# Autodesk Inventor assembly: Assembly1
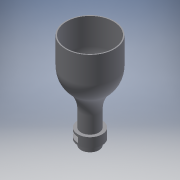
[picture p0: Inventor's stored thumbnail of the model, 180x180]
Saved by Autodesk Inventor 2018.3 (Build 223284000, 284)
## iProperties
Created: 2020-03-27
Part Number: Assembly1
Document SubType Name: Assembly
Designer: ToreDenStore
Author: ToreDenStore
## Documents named in this file (3)
- C:\Users\ToreDenStore\Documents\Inventor\Funnel wind turbine\Assembly1.iam
- C:\Users\ToreDenStore\Documents\Inventor\Funnel wind turbine\Outer tube.ipt
- C:\Users\ToreDenStore\Documents\Inventor\Funnel wind turbine\Rotator.ipt
## Components (2 placed, 2 different names)
1. Outer tube:1 — Rotational:1
2. Rotator:1 — Rotational:1
## Relationships (1: RevoluteJoint 1)
- Rotational:1 [RevoluteJoint]: Outer tube:1 ↔ Rotator:1
